# Autodesk Inventor assembly: camWithRubberBand
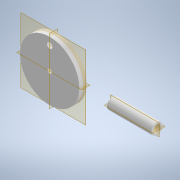
[picture p0: Inventor's stored thumbnail of the model, 180x180]
Saved by Autodesk Inventor 2020.2 (Build 242310000, 310)
## iProperties
Created: 2020-01-12
Part Number: camWithRubberBand
Document SubType Name: Assembly
Designer: robst
Author: robst
## Documents named in this file (3)
- C:\git\CAD-Development\robSteele\2020BallTriggerMechanism\camWithRubberBand.iam
- C:\git\CAD-Development\robSteele\2020LongRobotBase\camWheel.ipt
- C:\git\CAD-Development\robSteele\2020LongRobotBase\cylinderForKicker.ipt
## Components (2 placed, 2 different names)
1. camWheel:1 — Flush:1, Flush:2, Mate:1
2. cylinderForKicker:1 — Flush:1, Flush:2, Mate:1
## Relationships (3: Flush 2, Mate 1)
- Flush:1: camWheel:1 ↔ cylinderForKicker:1
- Flush:2: camWheel:1 ↔ cylinderForKicker:1
- Mate:1 (203.2 mm): camWheel:1 ↔ cylinderForKicker:1
